# Autodesk Inventor assembly: lightRingAssembly
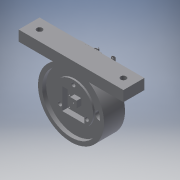
[picture p0: Inventor's stored thumbnail of the model, 180x180]
Saved by Autodesk Inventor 2019.3 (Build 233278000, 278)
## iProperties
Created: 2019-01-13
Part Number: lightRingAssembly
Document SubType Name: Assembly
Designer: steele
Author: steele
## Documents named in this file (5)
- C:\git\CAD-Development\robSteele\2019-FRC\sampleLightRingCameraMount\lightRingAssembly.iam
- C:\git\CAD-Development\robSteele\2019-FRC\sampleLightRingCameraMount\basicMount.ipt
- C:\git\CAD-Development\robSteele\ShapeWays\FRC\PiCameraAndLightRingMount\7712K620_BATTERY HOLDER.ipt
- C:\git\CAD-Development\robSteele\ShapeWays\FRC\PiCameraAndLightRingMount\MountCover.ipt
- C:\git\CAD-Development\robSteele\ShapeWays\FRC\PiCameraAndLightRingMount\RaspberryPiCameraModel.ipt
## Components (4 placed, 4 different names)
1. basicMount:1 — Mate:1, Flush:1, Flush:2, Insert:1, Insert:2
2. 7712K620_BATTERY HOLDER:1 — Mate:1, Flush:1, Flush:2
3. MountCover:1 — Insert:1
4. RaspberryPiCameraModel:1 — Insert:2
## Relationships (5: Flush 2, Insert 2, Mate 1)
- Mate:1: basicMount:1 ↔ 7712K620_BATTERY HOLDER:1
- Flush:1: basicMount:1 ↔ 7712K620_BATTERY HOLDER:1
- Flush:2: basicMount:1 ↔ 7712K620_BATTERY HOLDER:1
- Insert:1: basicMount:1 ↔ MountCover:1
- Insert:2: basicMount:1 ↔ RaspberryPiCameraModel:1
